# Autodesk Inventor assembly: 0.3rd Lawette - V3.0
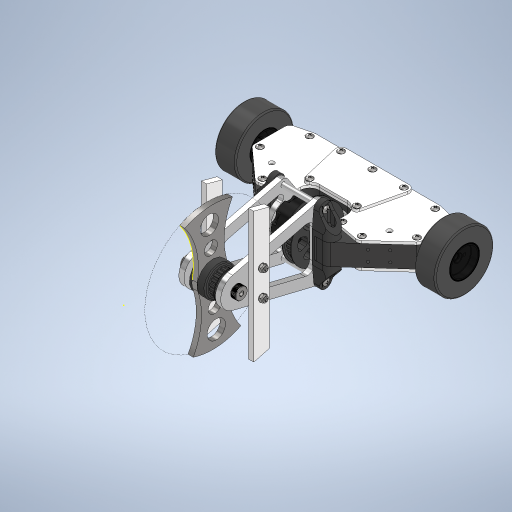
[picture p0: Inventor's stored thumbnail of the model, 512x512]
Saved by Autodesk Inventor 2023.1 (Build 271208000, 208)
## iProperties
Created: 2022-05-21
Part Number: 0.3rd Lawette - V3.0
Document SubType Name: Assembly
Designer: Nathan Cai
Mass: 1313 g
Surface Area: 3314.92 cm^2
Volume: 664.685 cm^3
Density: 1.97538 g/cm^3
Author: Nathan Cai
## Documents named in this file (21)
- E:\Documents\Inventor\0.3rd Lawette - V3.4\0.3rd Lawette - V3.4.iam
- E:\Documents\Inventor\0.3rd Lawette - V3.4\RR Brushless\RR-Brushless-Planetary.iam
- E:\Documents\Inventor\0.3rd Lawette - V3.4\Tattu 4S 650mah\Tattu 650mah 4S.iam
- E:\Documents\Inventor\0.3rd Lawette - V3.4\BL20A.ipt
- E:\Documents\Inventor\0.3rd Lawette - V3.4\Talon 25A ESC.ipt
- E:\Documents\Inventor\0.3rd Lawette - V3.4\Receiver (FrSky RX6R).ipt
- E:\Documents\Inventor\0.3rd Lawette - V3.4\Fingertech Power Switch\Fingertech Mini Power Switch.iam
- E:\Documents\Inventor\0.3rd Lawette - V3.4\Vertical Weapon Assembly\Weapon Assembly.iam
- E:\Documents\Inventor\0.3rd Lawette - V3.4\Chassis.ipt
- E:\Documents\Inventor\0.3rd Lawette - V3.4\Motor Plates.ipt
- E:\Documents\Inventor\0.3rd Lawette - V3.4\Motor Plates - Rear Insert.ipt
- E:\Documents\Inventor\0.3rd Lawette - V3.4\Standoff 1in.ipt
- E:\Documents\Inventor\0.3rd Lawette - V3.4\Cover (Inner Bottom).ipt
- E:\Documents\Inventor\0.3rd Lawette - V3.4\Cover (Inner Top).ipt
- E:\Documents\Inventor\0.3rd Lawette - V3.4\Cover (Outer).ipt
- E:\Documents\Inventor\Content Center Files\R2023\en-US\ANSI B18.6.3(27)\ANSI B18.6.3 - 6-32 UNC - 0.375(11).ipt
- E:\Documents\Inventor\Content Center Files\R2023\en-US\ANSI B18.6.3(27)\ANSI B18.6.3 - 6-32 UNC - 0.5(11).ipt
- E:\Documents\Inventor\0.3rd Lawette - V3.4\Botkit-Hubs.ipt
- E:\Documents\Inventor\0.3rd Lawette - V3.4\D2_Narrow_Wheels_2.75in_x_1in.ipt
- E:\Documents\Inventor\0.3rd Lawette - V3.4\Vertical Weapon Assembly (Type A)\Weapon Assembly (Vert A).iam
- E:\Documents\Inventor\0.3rd Lawette - V3.4\Horizontal Weapon Assembly (Type U)\Weapon Assembly (Horizontal U).iam
## Components (63 placed, 20 different names)
1. RR-Brushless-Planetary:1 [sub-assembly] — Mate:1, Flush:4, Mate:27, Mate:147, Mate:343, Mate:344
2. RR-Brushless-Planetary:2 [sub-assembly] — Mate:1, Flush:5, Mate:149, Mate:348, Mate:349
3. Tattu 650mah 4S:1 [sub-assembly] — Mate:15, Flush:9
4. BL20A:1 — Mate:2, Flush:1, Flush:2, Mate:14, Flush:7
5. BL20A:2 — Mate:2, Flush:1, Flush:2, Mate:3, Flush:3, Flush:8
6. Talon 25A ESC:1 — Mate:13, Flush:6, Mate:151
7. Receiver (FrSky RX6R):1 — Mate:3, Flush:3, Flush:8
8. Fingertech Mini Power Switch:1 [sub-assembly] — Flush:12, Mate:26, Mate:150
9. Chassis:1 — Flush:4, Flush:5, Mate:13, Flush:6, Mate:14, Flush:7, Mate:15, Flush:9, Flush:12, Mate:26, Mate:27, Mate:113, Mate:114, Mate:115, Mate:116, Mate:117, Mate:118, Mate:119, Mate:120, Mate:121, Mate:146, Flush:20, Mate:148, Flush:21, Mate:150, Mate:151, Mate:167, Mate:168, Mate:169, Mate:170, Mate:171, Mate:172, Mate:173, Mate:174, Mate:175, Mate:176, Mate:177, Flush:32, Mate:186, Mate:187, Mate:200, Mate:229, Mate:232, Mate:350, Mate:351, Mate:352, Mate:354, Mate:355, Mate:356
10. Motor Plates:1 — Mate:113, Mate:114, Mate:115
11. Motor Plates:2 — Mate:116, Mate:117, Mate:118
12. Motor Plates - Rear Insert:1 — Mate:146, Mate:147, Flush:20
13. Motor Plates - Rear Insert:2 — Mate:148, Mate:149, Flush:21
14. Standoff 1in:1 — Flush:22, Flush:23, Flush:24, Flush:25, Flush:26, Flush:27, Flush:28, Flush:29, Flush:30, Flush:31, Mate:167, Flush:32, Flush:33, Flush:34
15. Standoff 1in:2 — Flush:22, Mate:168
16. Standoff 1in:3 — Flush:25, Mate:175, Mate:233
17. Standoff 1in:4 — Flush:27, Mate:174
18. Standoff 1in:5 — Flush:29, Mate:173
19. Standoff 1in:6 — Flush:23, Mate:177
20. Standoff 1in:7 — Flush:24, Mate:176, Mate:231
21. Standoff 1in:8 — Flush:26, Mate:169
22. Standoff 1in:9 — Flush:28, Mate:170
23. Standoff 1in:10 — Flush:30, Mate:171, Mate:230
24. Standoff 1in:11 — Flush:31, Mate:172
25. Standoff 1in:12 — Mate:186, Flush:34
26. Standoff 1in:13 — Mate:187, Flush:33
27. Cover (Inner Bottom):1 — Mate:200, Mate:230, Mate:231, Mate:269, Mate:270, Mate:271, Mate:304, Mate:305, Mate:306, Mate:307, Mate:308, Mate:309, Mate:310, Mate:311, Mate:312, Mate:313, Mate:314, Mate:315, Mate:316, Mate:317, Mate:318, Mate:319
28. Cover (Inner Top):1 — Mate:229, Mate:232, Mate:233, Mate:266, Mate:267, Mate:268, Mate:288, Mate:289, Mate:290, Mate:291, Mate:292, Mate:293, Mate:294, Mate:295, Mate:296, Mate:297, Mate:298, Mate:299, Mate:300, Mate:301, Mate:302, Mate:303
29. Cover (Outer):1 — Mate:266, Mate:267, Mate:268, Mate:320, Mate:321, Mate:322, Mate:323, Mate:324, Mate:325, Mate:326, Mate:327, Mate:328, Mate:329
30. Cover (Outer):2 — Mate:269, Mate:270, Mate:271, Mate:330, Mate:331, Mate:332, Mate:333, Mate:334, Mate:335, Mate:336, Mate:337, Mate:338, Mate:339
31. Botkit-Hubs:1 — Mate:340, Mate:341, Mate:342, Mate:343, Mate:344
32. D2_Narrow_Wheels_2.75in_x_1in:1 — Mate:340, Mate:341, Mate:342
33. Botkit-Hubs:2 — Mate:345, Mate:346, Mate:347, Mate:348, Mate:349
34. D2_Narrow_Wheels_2.75in_x_1in:2 — Mate:345, Mate:346, Mate:347
35. Weapon Assembly (Vert A):1 [sub-assembly] — Mate:350, Mate:351, Mate:352
36. Weapon Assembly (Horizontal U):1 [sub-assembly] — Mate:354, Mate:355, Mate:356
37. Weapon Assembly:2 [sub-assembly] — Mate:119, Mate:120, Mate:121
38. Cross Recessed Truss Head Machine Screw - Type I - Inch No. 6 - 32 - 3/8:5 — Mate:288, Mate:289
39. Cross Recessed Truss Head Machine Screw - Type I - Inch No. 6 - 32 - 3/8:6 — Mate:290, Mate:291
40. Cross Recessed Truss Head Machine Screw - Type I - Inch No. 6 - 32 - 3/8:7 — Mate:292, Mate:293
41. Cross Recessed Truss Head Machine Screw - Type I - Inch No. 6 - 32 - 3/8:8 — Mate:294, Mate:295
42. Cross Recessed Truss Head Machine Screw - Type I - Inch No. 6 - 32 - 3/8:9 — Mate:296, Mate:297
43. Cross Recessed Truss Head Machine Screw - Type I - Inch No. 6 - 32 - 3/8:10 — Mate:298, Mate:299
44. Cross Recessed Truss Head Machine Screw - Type I - Inch No. 6 - 32 - 3/8:11 — Mate:300, Mate:301
45. Cross Recessed Truss Head Machine Screw - Type I - Inch No. 6 - 32 - 3/8:12 — Mate:302, Mate:303
46. Cross Recessed Truss Head Machine Screw - Type I - Inch No. 6 - 32 - 3/8:13 — Mate:304, Mate:305
47. Cross Recessed Truss Head Machine Screw - Type I - Inch No. 6 - 32 - 3/8:14 — Mate:306, Mate:307
48. Cross Recessed Truss Head Machine Screw - Type I - Inch No. 6 - 32 - 3/8:15 — Mate:308, Mate:309
49. Cross Recessed Truss Head Machine Screw - Type I - Inch No. 6 - 32 - 3/8:16 — Mate:310, Mate:311
50. Cross Recessed Truss Head Machine Screw - Type I - Inch No. 6 - 32 - 3/8:17 — Mate:312, Mate:313
51. Cross Recessed Truss Head Machine Screw - Type I - Inch No. 6 - 32 - 3/8:18 — Mate:314, Mate:315
52. Cross Recessed Truss Head Machine Screw - Type I - Inch No. 6 - 32 - 3/8:19 — Mate:316, Mate:317
53. Cross Recessed Truss Head Machine Screw - Type I - Inch No. 6 - 32 - 3/8:20 — Mate:318, Mate:319
54. Cross Recessed Truss Head Machine Screw - Type I - Inch No. 6 - 32 - 1/2:1 — Mate:320, Mate:321
55. Cross Recessed Truss Head Machine Screw - Type I - Inch No. 6 - 32 - 1/2:2 — Mate:322, Mate:323
56. Cross Recessed Truss Head Machine Screw - Type I - Inch No. 6 - 32 - 1/2:3 — Mate:324, Mate:325
57. Cross Recessed Truss Head Machine Screw - Type I - Inch No. 6 - 32 - 1/2:4 — Mate:326, Mate:327
58. Cross Recessed Truss Head Machine Screw - Type I - Inch No. 6 - 32 - 1/2:5 — Mate:328, Mate:329
59. Cross Recessed Truss Head Machine Screw - Type I - Inch No. 6 - 32 - 1/2:6 — Mate:330, Mate:331
60. Cross Recessed Truss Head Machine Screw - Type I - Inch No. 6 - 32 - 1/2:7 — Mate:332, Mate:333
61. Cross Recessed Truss Head Machine Screw - Type I - Inch No. 6 - 32 - 1/2:8 — Mate:334, Mate:335
62. Cross Recessed Truss Head Machine Screw - Type I - Inch No. 6 - 32 - 1/2:9 — Mate:336, Mate:337
63. Cross Recessed Truss Head Machine Screw - Type I - Inch No. 6 - 32 - 1/2:10 — Mate:338, Mate:339
## Relationships (141: Mate 116, Flush 25)
- Mate:1: RR-Brushless-Planetary:1 ↔ RR-Brushless-Planetary:2
- Mate:2: BL20A:1 ↔ BL20A:2
- Flush:1: BL20A:1 ↔ BL20A:2
- Flush:2: BL20A:1 ↔ BL20A:2
- Mate:3: BL20A:2 ↔ Receiver (FrSky RX6R):1
- Flush:3: BL20A:2 ↔ Receiver (FrSky RX6R):1
- Flush:4: RR-Brushless-Planetary:1 ↔ Chassis:1
- Flush:5: RR-Brushless-Planetary:2 ↔ Chassis:1
- Mate:13: Talon 25A ESC:1 ↔ Chassis:1
- Flush:6: Talon 25A ESC:1 ↔ Chassis:1
- Mate:14: BL20A:1 ↔ Chassis:1
- Flush:7: BL20A:1 ↔ Chassis:1
- Flush:8: BL20A:2 ↔ Receiver (FrSky RX6R):1
- Mate:15 (3.175 mm): Tattu 650mah 4S:1 ↔ Chassis:1
- Flush:9: Tattu 650mah 4S:1 ↔ Chassis:1
- Flush:12: Fingertech Mini Power Switch:1 ↔ Chassis:1
- Mate:26: Fingertech Mini Power Switch:1 ↔ Chassis:1
- Mate:27: RR-Brushless-Planetary:1 ↔ Chassis:1
- Mate:113: Chassis:1 ↔ Motor Plates:1
- Mate:114: Chassis:1 ↔ Motor Plates:1
- Mate:115: Chassis:1 ↔ Motor Plates:1
- Mate:116: Chassis:1 ↔ Motor Plates:2
- Mate:117: Chassis:1 ↔ Motor Plates:2
- Mate:118: Chassis:1 ↔ Motor Plates:2
- Mate:119: Chassis:1 ↔ Weapon Assembly:2
- Mate:120: Chassis:1 ↔ Weapon Assembly:2
- Mate:121 (9.525 mm): Chassis:1 ↔ Weapon Assembly:2
- Mate:146: Chassis:1 ↔ Motor Plates - Rear Insert:1
- Mate:147: RR-Brushless-Planetary:1 ↔ Motor Plates - Rear Insert:1
- Flush:20: Chassis:1 ↔ Motor Plates - Rear Insert:1
- Mate:148: Chassis:1 ↔ Motor Plates - Rear Insert:2
- Mate:149: RR-Brushless-Planetary:2 ↔ Motor Plates - Rear Insert:2
- Flush:21: Chassis:1 ↔ Motor Plates - Rear Insert:2
- Mate:150: Fingertech Mini Power Switch:1 ↔ Chassis:1
- Mate:151: Talon 25A ESC:1 ↔ Chassis:1
- Flush:22: Standoff 1in:1 ↔ Standoff 1in:2
- Flush:23: Standoff 1in:1 ↔ Standoff 1in:6
- Flush:24: Standoff 1in:1 ↔ Standoff 1in:7
- Flush:25: Standoff 1in:1 ↔ Standoff 1in:3
- Flush:26: Standoff 1in:1 ↔ Standoff 1in:8
- Flush:27: Standoff 1in:1 ↔ Standoff 1in:4
- Flush:28: Standoff 1in:1 ↔ Standoff 1in:9
- Flush:29: Standoff 1in:1 ↔ Standoff 1in:5
- Flush:30: Standoff 1in:1 ↔ Standoff 1in:10
- Flush:31: Standoff 1in:1 ↔ Standoff 1in:11
- Mate:167: Chassis:1 ↔ Standoff 1in:1
- Mate:168: Chassis:1 ↔ Standoff 1in:2
- Mate:169: Chassis:1 ↔ Standoff 1in:8
- Mate:170: Chassis:1 ↔ Standoff 1in:9
- Mate:171: Chassis:1 ↔ Standoff 1in:10
- Mate:172: Chassis:1 ↔ Standoff 1in:11
- Mate:173: Chassis:1 ↔ Standoff 1in:5
- Mate:174: Chassis:1 ↔ Standoff 1in:4
- Mate:175: Chassis:1 ↔ Standoff 1in:3
- Mate:176: Chassis:1 ↔ Standoff 1in:7
- Mate:177: Chassis:1 ↔ Standoff 1in:6
- Flush:32: Chassis:1 ↔ Standoff 1in:1
- Mate:186: Chassis:1 ↔ Standoff 1in:12
- Mate:187: Chassis:1 ↔ Standoff 1in:13
- Flush:33: Standoff 1in:1 ↔ Standoff 1in:13
- Flush:34: Standoff 1in:1 ↔ Standoff 1in:12
- Mate:200: Chassis:1 ↔ Cover (Inner Bottom):1
- Mate:229: Chassis:1 ↔ Cover (Inner Top):1
- Mate:230: Standoff 1in:10 ↔ Cover (Inner Bottom):1
- Mate:231: Standoff 1in:7 ↔ Cover (Inner Bottom):1
- Mate:232: Chassis:1 ↔ Cover (Inner Top):1
- Mate:233: Standoff 1in:3 ↔ Cover (Inner Top):1
- Mate:266: Cover (Inner Top):1 ↔ Cover (Outer):1
- Mate:267: Cover (Inner Top):1 ↔ Cover (Outer):1
- Mate:268: Cover (Inner Top):1 ↔ Cover (Outer):1
- Mate:269: Cover (Inner Bottom):1 ↔ Cover (Outer):2
- Mate:270: Cover (Inner Bottom):1 ↔ Cover (Outer):2
- Mate:271: Cover (Inner Bottom):1 ↔ Cover (Outer):2
- Mate:288: Cover (Inner Top):1 ↔ Cross Recessed Truss Head Machine Screw - Type I - Inch No. 6 - 32 - 3/8:5
- Mate:289: Cover (Inner Top):1 ↔ Cross Recessed Truss Head Machine Screw - Type I - Inch No. 6 - 32 - 3/8:5
- Mate:290: Cover (Inner Top):1 ↔ Cross Recessed Truss Head Machine Screw - Type I - Inch No. 6 - 32 - 3/8:6
- Mate:291: Cover (Inner Top):1 ↔ Cross Recessed Truss Head Machine Screw - Type I - Inch No. 6 - 32 - 3/8:6
- Mate:292: Cover (Inner Top):1 ↔ Cross Recessed Truss Head Machine Screw - Type I - Inch No. 6 - 32 - 3/8:7
- Mate:293: Cover (Inner Top):1 ↔ Cross Recessed Truss Head Machine Screw - Type I - Inch No. 6 - 32 - 3/8:7
- Mate:294: Cover (Inner Top):1 ↔ Cross Recessed Truss Head Machine Screw - Type I - Inch No. 6 - 32 - 3/8:8
- Mate:295: Cover (Inner Top):1 ↔ Cross Recessed Truss Head Machine Screw - Type I - Inch No. 6 - 32 - 3/8:8
- Mate:296: Cover (Inner Top):1 ↔ Cross Recessed Truss Head Machine Screw - Type I - Inch No. 6 - 32 - 3/8:9
- Mate:297: Cover (Inner Top):1 ↔ Cross Recessed Truss Head Machine Screw - Type I - Inch No. 6 - 32 - 3/8:9
- Mate:298: Cover (Inner Top):1 ↔ Cross Recessed Truss Head Machine Screw - Type I - Inch No. 6 - 32 - 3/8:10
- Mate:299: Cover (Inner Top):1 ↔ Cross Recessed Truss Head Machine Screw - Type I - Inch No. 6 - 32 - 3/8:10
- Mate:300: Cover (Inner Top):1 ↔ Cross Recessed Truss Head Machine Screw - Type I - Inch No. 6 - 32 - 3/8:11
- Mate:301: Cover (Inner Top):1 ↔ Cross Recessed Truss Head Machine Screw - Type I - Inch No. 6 - 32 - 3/8:11
- Mate:302: Cover (Inner Top):1 ↔ Cross Recessed Truss Head Machine Screw - Type I - Inch No. 6 - 32 - 3/8:12
- Mate:303: Cover (Inner Top):1 ↔ Cross Recessed Truss Head Machine Screw - Type I - Inch No. 6 - 32 - 3/8:12
- Mate:304: Cover (Inner Bottom):1 ↔ Cross Recessed Truss Head Machine Screw - Type I - Inch No. 6 - 32 - 3/8:13
- Mate:305: Cover (Inner Bottom):1 ↔ Cross Recessed Truss Head Machine Screw - Type I - Inch No. 6 - 32 - 3/8:13
- Mate:306: Cover (Inner Bottom):1 ↔ Cross Recessed Truss Head Machine Screw - Type I - Inch No. 6 - 32 - 3/8:14
- Mate:307: Cover (Inner Bottom):1 ↔ Cross Recessed Truss Head Machine Screw - Type I - Inch No. 6 - 32 - 3/8:14
- Mate:308: Cover (Inner Bottom):1 ↔ Cross Recessed Truss Head Machine Screw - Type I - Inch No. 6 - 32 - 3/8:15
- Mate:309: Cover (Inner Bottom):1 ↔ Cross Recessed Truss Head Machine Screw - Type I - Inch No. 6 - 32 - 3/8:15
- Mate:310: Cover (Inner Bottom):1 ↔ Cross Recessed Truss Head Machine Screw - Type I - Inch No. 6 - 32 - 3/8:16
- Mate:311: Cover (Inner Bottom):1 ↔ Cross Recessed Truss Head Machine Screw - Type I - Inch No. 6 - 32 - 3/8:16
- Mate:312: Cover (Inner Bottom):1 ↔ Cross Recessed Truss Head Machine Screw - Type I - Inch No. 6 - 32 - 3/8:17
- Mate:313: Cover (Inner Bottom):1 ↔ Cross Recessed Truss Head Machine Screw - Type I - Inch No. 6 - 32 - 3/8:17
- Mate:314: Cover (Inner Bottom):1 ↔ Cross Recessed Truss Head Machine Screw - Type I - Inch No. 6 - 32 - 3/8:18
- Mate:315: Cover (Inner Bottom):1 ↔ Cross Recessed Truss Head Machine Screw - Type I - Inch No. 6 - 32 - 3/8:18
- Mate:316: Cover (Inner Bottom):1 ↔ Cross Recessed Truss Head Machine Screw - Type I - Inch No. 6 - 32 - 3/8:19
- Mate:317: Cover (Inner Bottom):1 ↔ Cross Recessed Truss Head Machine Screw - Type I - Inch No. 6 - 32 - 3/8:19
- Mate:318: Cover (Inner Bottom):1 ↔ Cross Recessed Truss Head Machine Screw - Type I - Inch No. 6 - 32 - 3/8:20
- Mate:319: Cover (Inner Bottom):1 ↔ Cross Recessed Truss Head Machine Screw - Type I - Inch No. 6 - 32 - 3/8:20
- Mate:320: Cover (Outer):1 ↔ Cross Recessed Truss Head Machine Screw - Type I - Inch No. 6 - 32 - 1/2:1
- Mate:321: Cover (Outer):1 ↔ Cross Recessed Truss Head Machine Screw - Type I - Inch No. 6 - 32 - 1/2:1
- Mate:322: Cover (Outer):1 ↔ Cross Recessed Truss Head Machine Screw - Type I - Inch No. 6 - 32 - 1/2:2
- Mate:323: Cover (Outer):1 ↔ Cross Recessed Truss Head Machine Screw - Type I - Inch No. 6 - 32 - 1/2:2
- Mate:324: Cover (Outer):1 ↔ Cross Recessed Truss Head Machine Screw - Type I - Inch No. 6 - 32 - 1/2:3
- Mate:325: Cover (Outer):1 ↔ Cross Recessed Truss Head Machine Screw - Type I - Inch No. 6 - 32 - 1/2:3
- Mate:326: Cover (Outer):1 ↔ Cross Recessed Truss Head Machine Screw - Type I - Inch No. 6 - 32 - 1/2:4
- Mate:327: Cover (Outer):1 ↔ Cross Recessed Truss Head Machine Screw - Type I - Inch No. 6 - 32 - 1/2:4
- Mate:328: Cover (Outer):1 ↔ Cross Recessed Truss Head Machine Screw - Type I - Inch No. 6 - 32 - 1/2:5
- Mate:329: Cover (Outer):1 ↔ Cross Recessed Truss Head Machine Screw - Type I - Inch No. 6 - 32 - 1/2:5
- Mate:330: Cover (Outer):2 ↔ Cross Recessed Truss Head Machine Screw - Type I - Inch No. 6 - 32 - 1/2:6
- Mate:331: Cover (Outer):2 ↔ Cross Recessed Truss Head Machine Screw - Type I - Inch No. 6 - 32 - 1/2:6
- Mate:332: Cover (Outer):2 ↔ Cross Recessed Truss Head Machine Screw - Type I - Inch No. 6 - 32 - 1/2:7
- Mate:333: Cover (Outer):2 ↔ Cross Recessed Truss Head Machine Screw - Type I - Inch No. 6 - 32 - 1/2:7
- Mate:334: Cover (Outer):2 ↔ Cross Recessed Truss Head Machine Screw - Type I - Inch No. 6 - 32 - 1/2:8
- Mate:335: Cover (Outer):2 ↔ Cross Recessed Truss Head Machine Screw - Type I - Inch No. 6 - 32 - 1/2:8
- Mate:336: Cover (Outer):2 ↔ Cross Recessed Truss Head Machine Screw - Type I - Inch No. 6 - 32 - 1/2:9
- Mate:337: Cover (Outer):2 ↔ Cross Recessed Truss Head Machine Screw - Type I - Inch No. 6 - 32 - 1/2:9
- Mate:338: Cover (Outer):2 ↔ Cross Recessed Truss Head Machine Screw - Type I - Inch No. 6 - 32 - 1/2:10
- Mate:339: Cover (Outer):2 ↔ Cross Recessed Truss Head Machine Screw - Type I - Inch No. 6 - 32 - 1/2:10
- Mate:340: Botkit-Hubs:1 ↔ D2_Narrow_Wheels_2.75in_x_1in:1
- Mate:341: Botkit-Hubs:1 ↔ D2_Narrow_Wheels_2.75in_x_1in:1
- Mate:342: Botkit-Hubs:1 ↔ D2_Narrow_Wheels_2.75in_x_1in:1
- Mate:343: RR-Brushless-Planetary:1 ↔ Botkit-Hubs:1
- Mate:344 (-2 mm): RR-Brushless-Planetary:1 ↔ Botkit-Hubs:1
- Mate:345: Botkit-Hubs:2 ↔ D2_Narrow_Wheels_2.75in_x_1in:2
- Mate:346: Botkit-Hubs:2 ↔ D2_Narrow_Wheels_2.75in_x_1in:2
- Mate:347: Botkit-Hubs:2 ↔ D2_Narrow_Wheels_2.75in_x_1in:2
- Mate:348: RR-Brushless-Planetary:2 ↔ Botkit-Hubs:2
- Mate:349 (-2 mm): RR-Brushless-Planetary:2 ↔ Botkit-Hubs:2
- Mate:350: Chassis:1 ↔ Weapon Assembly (Vert A):1
- Mate:351: Chassis:1 ↔ Weapon Assembly (Vert A):1
- Mate:352: Chassis:1 ↔ Weapon Assembly (Vert A):1
- Mate:354: Chassis:1 ↔ Weapon Assembly (Horizontal U):1
- Mate:355: Chassis:1 ↔ Weapon Assembly (Horizontal U):1
- Mate:356: Chassis:1 ↔ Weapon Assembly (Horizontal U):1
